# Autodesk Inventor assembly: floor
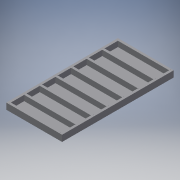
[picture p0: Inventor's stored thumbnail of the model, 180x180]
Saved by Autodesk Inventor 2017 (Build 210142000, 142)
## iProperties
Created: 2019-05-05
Part Number: floor
Document SubType Name: Assembly
Designer: Roman
Author: Roman
## Documents named in this file (4)
- C:\Users\Roman\Documents\CAD\tegu rev2\floor\floor.iam
- C:\Users\Roman\Documents\CAD\tegu rev2\floor\floor back.ipt
- C:\Users\Roman\Documents\CAD\tegu rev2\floor\floor long 2x4.ipt
- C:\Users\Roman\Documents\CAD\tegu rev2\floor\floor short 2x4.ipt
## Components (11 placed, 3 different names)
1. floor back:1 — Mate:1, Mate:2, Flush:1, Flush:2, Flush:3, Flush:4, Flush:5, Mate:4
2. floor long 2x4:1 — Mate:2, Flush:1, Flush:3
3. floor long 2x4:2 — Mate:1, Flush:2, Flush:4, Mate:3
4. floor short 2x4:1 — Mate:3, Flush:5, Mate:4
5. floor short 2x4:2
6. floor short 2x4:3
7. floor short 2x4:4
8. floor short 2x4:5
9. floor short 2x4:6
10. floor short 2x4:7
11. floor short 2x4:8
## Component patterns: (8 elements, first: floor short 2x4:1)
## Relationships (9: Flush 5, Mate 4)
- Mate:1: floor back:1 ↔ floor long 2x4:2
- Mate:2: floor back:1 ↔ floor long 2x4:1
- Flush:1: floor back:1 ↔ floor long 2x4:1
- Flush:2: floor back:1 ↔ floor long 2x4:2
- Flush:3: floor back:1 ↔ floor long 2x4:1
- Flush:4: floor back:1 ↔ floor long 2x4:2
- Mate:3: floor long 2x4:2 ↔ floor short 2x4:1
- Flush:5: floor back:1 ↔ floor short 2x4:1
- Mate:4: floor back:1 ↔ floor short 2x4:1
